# Autodesk Inventor assembly: assembly
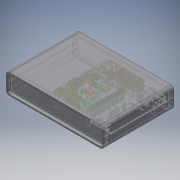
[picture p0: Inventor's stored thumbnail of the model, 180x180]
Saved by Autodesk Inventor 2017 (Build 210142000, 142)
## iProperties
Created: 2020-10-01
Part Number: assembly
Document SubType Name: Assembly
Designer: jferner
Author: jferner
## Documents named in this file (7)
- C:\dev\raspberry-pi-ir-hat\models3d\assembly.iam
- C:\dev\raspberry-pi-ir-hat\models3d\pcb\raspberry-pi-ir-hat.iam
- C:\dev\raspberry-pi-ir-hat\models3d\raspberry-pi-3\Raspberry Pi 3.iam
- C:\dev\raspberry-pi-ir-hat\models3d\case\case-bottom.ipt
- C:\dev\raspberry-pi-ir-hat\models3d\case\case-back.ipt
- C:\dev\raspberry-pi-ir-hat\models3d\case\case-front.ipt
- C:\dev\raspberry-pi-ir-hat\models3d\case\case-top.ipt
## Components (6 placed, 6 different names)
1. Raspberry Pi 3:1 [sub-assembly] — Mate:1, Flush:1, Flush:2, Mate:5, Mate:6, Mate:7
2. raspberry-pi-ir-hat:1 [sub-assembly] — Mate:1, Flush:1, Flush:2
3. case-bottom:1 — Mate:8, Mate:9, Mate:10, Mate:11, Mate:12, Mate:13
4. case-back:1 — Mate:5, Mate:6, Mate:7, Mate:11, Mate:12, Mate:13, Mate:14, Mate:15, Mate:16
5. case-front:1 — Mate:8, Mate:9, Mate:10
6. case-top:1 — Mate:14, Mate:15, Mate:16
## Relationships (15: Mate 13, Flush 2)
- Mate:1: Raspberry Pi 3:1 ↔ raspberry-pi-ir-hat:1
- Flush:1: Raspberry Pi 3:1 ↔ raspberry-pi-ir-hat:1
- Flush:2: Raspberry Pi 3:1 ↔ raspberry-pi-ir-hat:1
- Mate:5 (0.5 mm): Raspberry Pi 3:1 ↔ case-back:1
- Mate:6 (0.5 mm): Raspberry Pi 3:1 ↔ case-back:1
- Mate:7 (0.5 mm): Raspberry Pi 3:1 ↔ case-back:1
- Mate:8: case-bottom:1 ↔ case-front:1
- Mate:9: case-bottom:1 ↔ case-front:1
- Mate:10: case-bottom:1 ↔ case-front:1
- Mate:11: case-bottom:1 ↔ case-back:1
- Mate:12: case-bottom:1 ↔ case-back:1
- Mate:13: case-bottom:1 ↔ case-back:1
- Mate:14: case-back:1 ↔ case-top:1
- Mate:15: case-back:1 ↔ case-top:1
- Mate:16: case-back:1 ↔ case-top:1
